# Autodesk Inventor assembly: prototipo
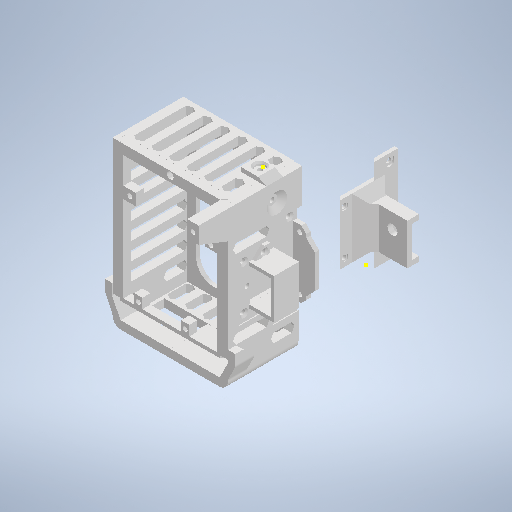
[picture p0: Inventor's stored thumbnail of the model, 512x512]
Saved by Autodesk Inventor 2025.1 (Build 291241000, 241)
## iProperties
Created: 2024-03-02
Part Number: prototipo
Document SubType Name: Assembly
Designer: joaov
Author: joaov
## Documents named in this file (9)
- C:\Joao_backup\bancada_arduino_uno\bancada_arduino_uno.iam
- C:\Joao_backup\bancada_arduino_uno\corpo.ipt
- C:\Joao_backup\bancada_arduino_uno\tampa.ipt
- C:\Joao_backup\bancada_arduino_uno\ventilador.ipt
- C:\Joao_backup\bancada_arduino_uno\protetor_luz.ipt
- C:\Joao_backup\bancada_arduino_uno\suporte_esquerdo.ipt
- C:\Joao_backup\bancada_arduino_uno\porta.ipt
- C:\Joao_backup\bancada_arduino_uno\porta_MIR.ipt
- C:\Joao_backup\bancada_arduino_uno\ventilador_CPY.ipt
## Components (8 placed, 8 different names)
1. corpo:1 — Coincidente:2, Coincidente:3, Alinhado:3, Coincidente:4, Coincidente:13, Coincidente:14, Coincidente:15, Coincidente:16
2. tampa_1 — Coincidente:2, Coincidente:3
3. ventilador:1 — Coincidente:7, Coincidente:8, Coincidente:15
4. protetor_luz:1 — Coincidente:7, Coincidente:8
5. suporte_esquerdo:1 — Alinhado:3, Coincidente:4, Coincidente:16
6. porta:1 — Coincidente:11, Coincidente:12, Coincidente:14
7. porta_MIR:1 — Coincidente:11, Coincidente:12, Coincidente:13
8. bloco_aquecimento
## Relationships (12: Mate 11, Flush 1)
- Coincidente:2 [Mate]: corpo:1 ↔ tampa_1
- Coincidente:3 [Mate]: corpo:1 ↔ tampa_1
- Alinhado:3 [Flush]: corpo:1 ↔ suporte_esquerdo:1
- Coincidente:4 [Mate]: corpo:1 ↔ suporte_esquerdo:1
- Coincidente:7 [Mate]: ventilador:1 ↔ protetor_luz:1
- Coincidente:8 [Mate]: ventilador:1 ↔ protetor_luz:1
- Coincidente:11 [Mate]: porta:1 ↔ porta_MIR:1
- Coincidente:12 [Mate]: porta:1 ↔ porta_MIR:1
- Coincidente:13 [Mate]: corpo:1 ↔ porta_MIR:1
- Coincidente:14 [Mate]: corpo:1 ↔ porta:1
- Coincidente:15 [Mate]: corpo:1 ↔ ventilador:1
- Coincidente:16 [Mate]: corpo:1 ↔ suporte_esquerdo:1
